# Autodesk Inventor assembly: 3-6V DC Gearbox Electromotor_MIR
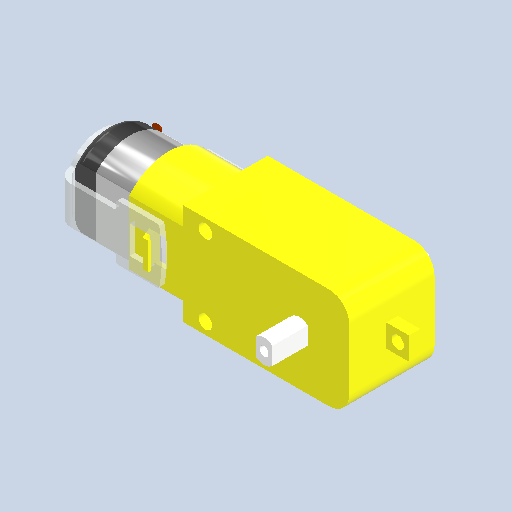
[picture p0: Inventor's stored thumbnail of the model, 512x512]
Saved by Autodesk Inventor 2023 (Build 270158000, 158)
## iProperties
Created: 2020-10-26
Part Number: 3-6V DC Gearbox Electromotor_MIR
Document SubType Name: Assembly
Designer: ASUS
Author: Niels
## Documents named in this file (4)
- D:\Backup C\Documents\Inventor\PMLDCAPSTONE\Gearbox\3-6V DC Gearbox Electromotor_MIR.iam
- D:\Backup C\Documents\Inventor\PMLDCAPSTONE\Gearbox\DC 3-6V Gearbox Motor_MIR.ipt
- D:\Backup C\Documents\Inventor\PMLDCAPSTONE\Gearbox\3V DC Electromotor_MIR.ipt
- D:\Backup C\Documents\Inventor\PMLDCAPSTONE\Gearbox\Part3 - Gearbox_MIR.ipt
## Components (3 placed, 3 different names)
1. DC 3-6V Gearbox Motor_MIR:1 — Mate:1, Insert:1, Flush:1
2. 3V DC Electromotor_MIR:1 — Mate:1, Insert:1
3. Part3 - Gearbox_MIR:1 — Flush:2
## Relationships (4: Mate 2, Insert 1, Flush 1)
- Mate:1 (0.15 mm): DC 3-6V Gearbox Motor_MIR:1 ↔ 3V DC Electromotor_MIR:1
- Insert:1: DC 3-6V Gearbox Motor_MIR:1 ↔ 3V DC Electromotor_MIR:1
- Flush:2 [Mate]: Part3 - Gearbox_MIR:1
- Flush:1 (-3 mm): DC 3-6V Gearbox Motor_MIR:1
